# Autodesk Inventor assembly: 2016 Chassie with 2018 Gearbox
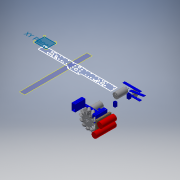
[picture p0: Inventor's stored thumbnail of the model, 180x180]
Saved by Autodesk Inventor 2018 (Build 220112000, 112)
## iProperties
Created: 2018-01-16
Part Number: 2016 Chassie with 2018 Gearbox
Document SubType Name: Assembly
Designer: Apple
Author: Apple
## Documents named in this file (18)
- C:\Users\Apple\Documents\Inventor\2018 PowerUp\2016 Chassie with 2018 Gearbox.iam
- C:\Users\Apple\Documents\Inventor\2018 PowerUp\2016 plate with 2018 boxes.iam
- C:\Users\Apple\Documents\Inventor\2018 PowerUp\2016_Files_2018_Mod\Assembly\Imported Components\My2 am-2953 AM14U2 End Sheet Square.ipt.ipt
- C:\Users\Apple\Documents\Inventor\2018 PowerUp\2016_Files_2018_Mod\Assembly\Imported Components\My2 am-2953 AM14U2 End Sheet Square Intake.ipt
- C:\Users\Apple\Documents\Inventor\2018 PowerUp\Bumper\Side Bumper.iam
- C:\Users\Apple\Documents\Inventor\2018 PowerUp\Bumper\Intake Bumper1.iam
- C:\Users\Apple\Documents\Inventor\2018 PowerUp\Bumper\Front Bumper1.iam
- C:\Users\Apple\Documents\Inventor\2018 PowerUp\2018 Cube Backstop Mount.ipt
- C:\Users\Apple\Documents\Inventor\2018 PowerUp\2018 Cube Back Stop Top_Botom.ipt
- C:\Users\Apple\Documents\Inventor\2018 PowerUp\2018 Cube Back Stop Vertical.ipt
- C:\Users\Apple\Documents\Inventor\2018 PowerUp\2018 Scissor\2018 Scissor Standoff Iner.ipt
- C:\Users\Apple\Documents\Inventor\2018 PowerUp\2018 Scissor\2018 Scissor Stand Off Outside A.ipt
- C:\Users\Apple\Documents\Inventor\2018 PowerUp\2018 Scissor\2018 Scissor Stand Off Outside B.ipt
- C:\Users\Apple\Documents\Inventor\2018 PowerUp\2018 Cube Backstop Mount Angle.ipt
- C:\Users\Apple\Documents\Inventor\2018 PowerUp\2018 Top Cross Bar.ipt
- C:\Users\Apple\Documents\Inventor\2018 PowerUp\2018 Bottom Cross Bar.ipt
- C:\Users\Apple\Documents\Inventor\2018 PowerUp\Winch\Winch Concept.iam
- My2 am-2953 AM14U2 End Sheet Square.ipt
## Components (32 placed, 16 different names)
1. 2016 plate with 2018 boxes:1 [sub-assembly] — Flush:1, Flush:2, Mate:12, Bumper Height, Mate:15, Mate:16, Flush:23, Flush:24, Mate:24, Mate:6, Mate:25, Mate:29, Mate:30, Angle:2, Mate:31, Mate:32, Angle:3, Angle:5, Mate:47, Mate:48
2. 2016 plate with 2018 boxes:2 [sub-assembly] — Flush:1, Flush:2, Mate:1, Mate:13, Flush:18, Mate:17, Flush:22, Flush:25, Flush:26, Mate:23, Mate:26, Mate:27, Mate:28, Angle:1, Mate:33, Mate:34, Angle:4, Angle:6, Mate:45, Mate:46
3. My2 am-2953 AM14U2 End Sheet Square.ipt:1 — Mate:1, Mate:14, Mate:23, Mate:24, Mate:35, Mate:36, Mate:39, Mate:40, Angle:7, Mate:51, Mate:52
4. My2 am-2953 AM14U2 End Sheet Square Intake:1 — Mate:6, Mate:25, Mate:26, Mate:37, Mate:38, Mate:41, Mate:42, Angle:8, Flush:36, Mate:43, Mate:44
5. 2018 Top Cross Bar:1 — Mate:45, Mate:46
6. 2018 Bottom Cross Bar:1 — Mate:47, Mate:48
7. Winch Concept:1 [sub-assembly] — Mate:51, Mate:52
8. 2018 Cube Backstop Mount Angle:2 — Mate:43, Mate:44
9. 2018 Cube Backstop Mount Angle:1 — Flush:36
10. 2018 Cube Backstop Mount:2 — Mate:16, Flush:19, Flush:20, Flush:24, Mate:19
11. 2018 Cube Backstop Mount:3 — Mate:17, Flush:19, Flush:21, Flush:26
12. 2018 Cube Backstop Mount:4 — Mate:15, Flush:20, Flush:23, Flush:28, Mate:18
13. 2018 Cube Back Stop Top_Botom:1 — Flush:27, Flush:28, Mate:18, Flush:29, Flush:30, Flush:31, Flush:34, Mate:20, Mate:21
14. 2018 Cube Back Stop Top_Botom:2 — Mate:19, Flush:29, Flush:30, Flush:35
15. 2018 Cube Back Stop Vertical:1 — Flush:31, Flush:32, Mate:22
16. 2018 Cube Back Stop Vertical:2 — Flush:32, Flush:33, Flush:34, Mate:21, Flush:35
17. 2018 Cube Back Stop Vertical:3 — Flush:33, Mate:20, Mate:22
18. 2018 Cube Backstop Mount:1 — Flush:18, Flush:21, Flush:22, Flush:25, Flush:27
19. 2018 Scissor Standoff Iner:1 — Mate:27, Mate:28, Angle:1
20. 2018 Scissor Standoff Iner:2 — Mate:29, Mate:30, Angle:2
21. 2018 Scissor Standoff Iner:3 — Mate:31, Mate:32, Angle:3
22. 2018 Scissor Standoff Iner:4 — Mate:33, Mate:34, Angle:4
23. 2018 Scissor Stand Off Outside A:1 — Mate:35, Mate:36, Angle:6
24. 2018 Scissor Stand Off Outside A:2 — Mate:37, Mate:38, Angle:5
25. 2018 Scissor Stand Off Outside B:1 — Mate:41, Mate:42, Angle:8
26. 2018 Scissor Stand Off Outside B:2 — Mate:39, Mate:40, Angle:7
27. Side Bumper:1 [sub-assembly] — Mate:7, Flush:5, Flush:6, Flush:9, Flush:12, Mate:10, Flush:13, Mate:13
28. Side Bumper:2 [sub-assembly] — Flush:7, Mate:8, Flush:8, Flush:9, Mate:11, Flush:14, Flush:15, Mate:12, Bumper Height
29. Intake Bumper1:1 [sub-assembly] — Flush:7, Mate:8, Flush:8
30. Intake Bumper1:2 [sub-assembly] — Mate:7, Flush:5, Flush:6
31. Front Bumper1:2 [sub-assembly] — Flush:12, Mate:10, Flush:13, Flush:16, Mate:14
32. Front Bumper1:3 [sub-assembly] — Mate:11, Flush:14, Flush:15, Flush:16
## Relationships (87: Mate 46, Flush 33, Angle 8)
- Flush:1: 2016 plate with 2018 boxes:1 ↔ 2016 plate with 2018 boxes:2
- Flush:2: 2016 plate with 2018 boxes:1 ↔ 2016 plate with 2018 boxes:2
- Mate:1: 2016 plate with 2018 boxes:2 ↔ My2 am-2953 AM14U2 End Sheet Square.ipt:1
- Mate:6: 2016 plate with 2018 boxes:1 ↔ My2 am-2953 AM14U2 End Sheet Square Intake:1
- Mate:7: Side Bumper:1 ↔ Intake Bumper1:2
- Flush:5: Side Bumper:1 ↔ Intake Bumper1:2
- Flush:6: Side Bumper:1 ↔ Intake Bumper1:2
- Flush:7: Side Bumper:2 ↔ Intake Bumper1:1
- Mate:8: Side Bumper:2 ↔ Intake Bumper1:1
- Flush:8: Side Bumper:2 ↔ Intake Bumper1:1
- Flush:9: Side Bumper:1 ↔ Side Bumper:2
- Flush:12: Side Bumper:1 ↔ Front Bumper1:2
- Mate:10: Side Bumper:1 ↔ Front Bumper1:2
- Flush:13: Side Bumper:1 ↔ Front Bumper1:2
- Mate:11 (2 mm): Side Bumper:2 ↔ Front Bumper1:3
- Flush:14: Side Bumper:2 ↔ Front Bumper1:3
- Flush:15: Side Bumper:2 ↔ Front Bumper1:3
- Mate:12 (0.0049 mm): 2016 plate with 2018 boxes:1 ↔ Side Bumper:2
- Mate:13 (2 mm): 2016 plate with 2018 boxes:2 ↔ Side Bumper:1
- Flush:16: Front Bumper1:2 ↔ Front Bumper1:3
- Mate:14: My2 am-2953 AM14U2 End Sheet Square.ipt:1 ↔ Front Bumper1:2
- Bumper Height [Flush] (50 mm): 2016 plate with 2018 boxes:1 ↔ Side Bumper:2
- Flush:18: 2016 plate with 2018 boxes:2 ↔ 2018 Cube Backstop Mount:1
- Mate:15: 2016 plate with 2018 boxes:1 ↔ 2018 Cube Backstop Mount:4
- Mate:16: 2016 plate with 2018 boxes:1 ↔ 2018 Cube Backstop Mount:2
- Mate:17: 2016 plate with 2018 boxes:2 ↔ 2018 Cube Backstop Mount:3
- Flush:19: 2018 Cube Backstop Mount:2 ↔ 2018 Cube Backstop Mount:3
- Flush:20: 2018 Cube Backstop Mount:2 ↔ 2018 Cube Backstop Mount:4
- Flush:21: 2018 Cube Backstop Mount:3 ↔ 2018 Cube Backstop Mount:1
- Flush:22: 2016 plate with 2018 boxes:2 ↔ 2018 Cube Backstop Mount:1
- Flush:23: 2016 plate with 2018 boxes:1 ↔ 2018 Cube Backstop Mount:4
- Flush:24: 2016 plate with 2018 boxes:1 ↔ 2018 Cube Backstop Mount:2
- Flush:25: 2016 plate with 2018 boxes:2 ↔ 2018 Cube Backstop Mount:1
- Flush:26: 2016 plate with 2018 boxes:2 ↔ 2018 Cube Backstop Mount:3
- Flush:27: 2018 Cube Back Stop Top_Botom:1 ↔ 2018 Cube Backstop Mount:1
- Flush:28 (55 mm): 2018 Cube Backstop Mount:4 ↔ 2018 Cube Back Stop Top_Botom:1
- Mate:18: 2018 Cube Backstop Mount:4 ↔ 2018 Cube Back Stop Top_Botom:1
- Mate:19: 2018 Cube Backstop Mount:2 ↔ 2018 Cube Back Stop Top_Botom:2
- Flush:29: 2018 Cube Back Stop Top_Botom:1 ↔ 2018 Cube Back Stop Top_Botom:2
- Flush:30: 2018 Cube Back Stop Top_Botom:1 ↔ 2018 Cube Back Stop Top_Botom:2
- Flush:31: 2018 Cube Back Stop Top_Botom:1 ↔ 2018 Cube Back Stop Vertical:1
- Flush:32: 2018 Cube Back Stop Vertical:1 ↔ 2018 Cube Back Stop Vertical:2
- Flush:33: 2018 Cube Back Stop Vertical:2 ↔ 2018 Cube Back Stop Vertical:3
- Flush:34: 2018 Cube Back Stop Top_Botom:1 ↔ 2018 Cube Back Stop Vertical:2
- Mate:20: 2018 Cube Back Stop Top_Botom:1 ↔ 2018 Cube Back Stop Vertical:3
- Mate:21: 2018 Cube Back Stop Top_Botom:1 ↔ 2018 Cube Back Stop Vertical:2
- Flush:35: 2018 Cube Back Stop Top_Botom:2 ↔ 2018 Cube Back Stop Vertical:2
- Mate:22 (129 mm): 2018 Cube Back Stop Vertical:1 ↔ 2018 Cube Back Stop Vertical:3
- Mate:23: 2016 plate with 2018 boxes:2 ↔ My2 am-2953 AM14U2 End Sheet Square.ipt:1
- Mate:24: 2016 plate with 2018 boxes:1 ↔ My2 am-2953 AM14U2 End Sheet Square.ipt:1
- Mate:25: 2016 plate with 2018 boxes:1 ↔ My2 am-2953 AM14U2 End Sheet Square Intake:1
- Mate:26: 2016 plate with 2018 boxes:2 ↔ My2 am-2953 AM14U2 End Sheet Square Intake:1
- Mate:27: 2016 plate with 2018 boxes:2 ↔ 2018 Scissor Standoff Iner:1
- Mate:28: 2016 plate with 2018 boxes:2 ↔ 2018 Scissor Standoff Iner:1
- Angle:1 (90 deg): 2016 plate with 2018 boxes:2 ↔ 2018 Scissor Standoff Iner:1
- Mate:29: 2016 plate with 2018 boxes:1 ↔ 2018 Scissor Standoff Iner:2
- Mate:30: 2016 plate with 2018 boxes:1 ↔ 2018 Scissor Standoff Iner:2
- Angle:2 (270 deg): 2016 plate with 2018 boxes:1 ↔ 2018 Scissor Standoff Iner:2
- Mate:31: 2016 plate with 2018 boxes:1 ↔ 2018 Scissor Standoff Iner:3
- Mate:32: 2016 plate with 2018 boxes:1 ↔ 2018 Scissor Standoff Iner:3
- Angle:3 (270 deg): 2016 plate with 2018 boxes:1 ↔ 2018 Scissor Standoff Iner:3
- Mate:33: 2016 plate with 2018 boxes:2 ↔ 2018 Scissor Standoff Iner:4
- Mate:34: 2016 plate with 2018 boxes:2 ↔ 2018 Scissor Standoff Iner:4
- Angle:4 (0 deg): 2016 plate with 2018 boxes:2 ↔ 2018 Scissor Standoff Iner:4
- Mate:35: My2 am-2953 AM14U2 End Sheet Square.ipt:1 ↔ 2018 Scissor Stand Off Outside A:1
- Mate:36: My2 am-2953 AM14U2 End Sheet Square.ipt:1 ↔ 2018 Scissor Stand Off Outside A:1
- Mate:37: My2 am-2953 AM14U2 End Sheet Square Intake:1 ↔ 2018 Scissor Stand Off Outside A:2
- Mate:38: My2 am-2953 AM14U2 End Sheet Square Intake:1 ↔ 2018 Scissor Stand Off Outside A:2
- Angle:5 (270 deg): 2016 plate with 2018 boxes:1 ↔ 2018 Scissor Stand Off Outside A:2
- Angle:6 (270 deg): 2016 plate with 2018 boxes:2 ↔ 2018 Scissor Stand Off Outside A:1
- Mate:39: My2 am-2953 AM14U2 End Sheet Square.ipt:1 ↔ 2018 Scissor Stand Off Outside B:2
- Mate:40: My2 am-2953 AM14U2 End Sheet Square.ipt:1 ↔ 2018 Scissor Stand Off Outside B:2
- Angle:7 (0 deg): My2 am-2953 AM14U2 End Sheet Square.ipt:1 ↔ 2018 Scissor Stand Off Outside B:2
- Mate:41: My2 am-2953 AM14U2 End Sheet Square Intake:1 ↔ 2018 Scissor Stand Off Outside B:1
- Mate:42: My2 am-2953 AM14U2 End Sheet Square Intake:1 ↔ 2018 Scissor Stand Off Outside B:1
- Angle:8 (0 deg): My2 am-2953 AM14U2 End Sheet Square Intake:1 ↔ 2018 Scissor Stand Off Outside B:1
- Flush:36: My2 am-2953 AM14U2 End Sheet Square Intake:1 ↔ 2018 Cube Backstop Mount Angle:1
- Mate:43: My2 am-2953 AM14U2 End Sheet Square Intake:1 ↔ 2018 Cube Backstop Mount Angle:2
- Mate:44: My2 am-2953 AM14U2 End Sheet Square Intake:1 ↔ 2018 Cube Backstop Mount Angle:2
- Mate:45: 2016 plate with 2018 boxes:2 ↔ 2018 Top Cross Bar:1
- Mate:46: 2016 plate with 2018 boxes:2 ↔ 2018 Top Cross Bar:1
- Mate:47: 2016 plate with 2018 boxes:1 ↔ 2018 Bottom Cross Bar:1
- Mate:48: 2016 plate with 2018 boxes:1 ↔ 2018 Bottom Cross Bar:1
- [Flush] (50 mm): 2016 plate with 2018 boxes:1 ↔ Winch Concept:1
- [Mate] (50 mm): 2016 plate with 2018 boxes:2 ↔ Winch Concept:1
- Mate:51: My2 am-2953 AM14U2 End Sheet Square.ipt:1 ↔ Winch Concept:1
- Mate:52: My2 am-2953 AM14U2 End Sheet Square.ipt:1 ↔ Winch Concept:1
